# Autodesk Inventor assembly: A_Airbert
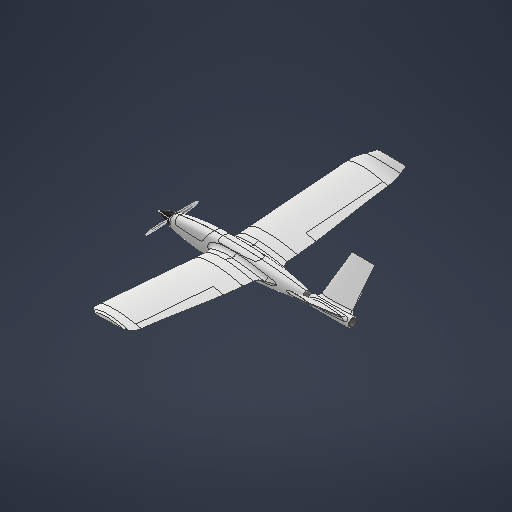
[picture p0: Inventor's stored thumbnail of the model, 512x512]
Saved by Autodesk Inventor 2026 (Build 300175000, 175)
## iProperties
Created: 2025-08-22
Part Number: A_Airbert
Document SubType Name: Assembly
Designer: FAL
Mass: 1462.69 g
Surface Area: 5659.36 cm^2
Volume: 1893.44 cm^3
Author: FAL
## Documents named in this file (11)
- C:\Users\FAL\Projekte\Git\AEROLAB\01_AIRCRAFTS\Airbert\A_Airbert.iam
- C:\Users\FAL\Projekte\Git\AEROLAB\01_AIRCRAFTS\Airbert\P_Fuselage.ipt
- C:\Users\FAL\Projekte\Git\AEROLAB\01_AIRCRAFTS\Airbert\P_MotorNose.ipt
- C:\Users\FAL\Projekte\Git\AEROLAB\01_AIRCRAFTS\Airbert\P_Carbon_Pipe_Back.ipt
- C:\Users\FAL\Projekte\Git\AEROLAB\01_AIRCRAFTS\Airbert\extern\P_AP-PR-006_6-2_LH.ipt
- C:\Users\FAL\Projekte\Git\AEROLAB\01_AIRCRAFTS\Airbert\P_Heck.ipt
- C:\Users\FAL\Projekte\Git\AEROLAB\01_AIRCRAFTS\Airbert\extern\P_Akku_Dummy.ipt
- C:\Users\FAL\Projekte\Git\AEROLAB\01_AIRCRAFTS\Airbert\P_Heck_T.ipt
- C:\Users\FAL\Projekte\Git\AEROLAB\01_AIRCRAFTS\Airbert\extern\P_BLDC_2200KV.ipt
- C:\Users\FAL\Projekte\Git\AEROLAB\01_AIRCRAFTS\Airbert\extern\P_Receiver_Radiolink.ipt
- C:\Users\FAL\Projekte\Git\AEROLAB\01_AIRCRAFTS\Airbert\extern\P_ESC_40A.ipt
## Components (10 placed, 10 different names)
1. P_Fuselage:1 — Fluchtend:1, Fluchtend:2, Fluchtend:3, Passend:1, Passend:2, Passend:8
2. P_MotorNose:1 — Passend:1, Passend:2, Passend:5, Passend:11
3. P_Carbon_Pipe_Back:1 — Passend:6, Passend:8, Fluchtend:9, Passend:10, Fluchtend:10
4. P_AP-PR-006_6-2_LH:1 — Passend:5
5. P_Akku_Dummy:1 — Passend:7
6. P_BLDC_2200KV:1 — Passend:11
7. P_Receiver_Radiolink:1
8. P_ESC_40A:1
9. P_Heck:1 — Passend:6, Fluchtend:8, Fluchtend:9
10. P_Heck_T:1 — Passend:9, Passend:10, Fluchtend:10
## Relationships (15: Mate 9, Flush 6)
- Fluchtend:1 [Flush]: P_Fuselage:1
- Fluchtend:2 [Flush]: P_Fuselage:1
- Fluchtend:3 [Flush]: P_Fuselage:1
- Passend:1 [Mate]: P_Fuselage:1 ↔ P_MotorNose:1
- Passend:2 [Mate]: P_Fuselage:1 ↔ P_MotorNose:1
- Passend:5 [Mate]: P_MotorNose:1 ↔ P_AP-PR-006_6-2_LH:1
- Passend:6 [Mate]: P_Carbon_Pipe_Back:1 ↔ P_Heck:1
- Fluchtend:8 [Flush]: P_Heck:1
- Passend:7 [Mate]: P_Akku_Dummy:1
- Passend:8 [Mate]: P_Fuselage:1 ↔ P_Carbon_Pipe_Back:1
- Fluchtend:9 [Flush]: P_Carbon_Pipe_Back:1 ↔ P_Heck:1
- Passend:9 [Mate]: P_Heck_T:1
- Passend:10 [Mate]: P_Carbon_Pipe_Back:1 ↔ P_Heck_T:1
- Fluchtend:10 [Flush]: P_Carbon_Pipe_Back:1 ↔ P_Heck_T:1
- Passend:11 [Mate]: P_MotorNose:1 ↔ P_BLDC_2200KV:1
